# Autodesk Inventor assembly: TopPlate
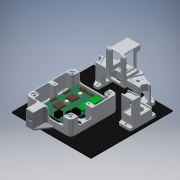
[picture p0: Inventor's stored thumbnail of the model, 180x180]
Saved by Autodesk Inventor 2016 (Build 200138000, 138)
## iProperties
Created: 2015-08-28
Part Number: TopPlate
Document SubType Name: Assembly
Designer: lachesis
Author: lachesis
## Documents named in this file (6)
- C:\Users\lachesis\git\Swarmie-Build\Swarmie-Assembly\Assemblies\TopPlate.iam
- C:\Users\lachesis\git\Swarmie-Build\Swarmie-Assembly\Parts\TopPlate.ipt
- C:\Users\lachesis\git\Swarmie-Build\Swarmie-Assembly\Parts\USTowerLW.ipt
- C:\Users\lachesis\git\Swarmie-Build\Swarmie-Assembly\Parts\CameraMountLW.ipt
- C:\Users\lachesis\git\Swarmie-Build\Swarmie-Assembly\Parts\GPS_IMUMountLW.ipt
- C:\Users\lachesis\git\Swarmie-Build\Swarmie-Assembly\Assemblies\NUCBase-PCB.iam
## Components (5 placed, 5 different names)
1. TopPlate:1 — Rigid:2, Rigid:5, Rigid:7
2. GPS_IMUMountLW:1 — Rigid:2
3. USTowerLW:1 — Rigid:5, Rigid:6
4. CameraMountLW:1 — Rigid:6
5. NUCBase-PCB:1 [sub-assembly] — Rigid:7
## Relationships (4: WeldJoint 4)
- Rigid:2 [WeldJoint]: TopPlate:1 ↔ GPS_IMUMountLW:1
- Rigid:5 [WeldJoint]: TopPlate:1 ↔ USTowerLW:1
- Rigid:6 [WeldJoint]: USTowerLW:1 ↔ CameraMountLW:1
- Rigid:7 [WeldJoint]: TopPlate:1 ↔ NUCBase-PCB:1
